# Autodesk Inventor assembly: Сборка ручка
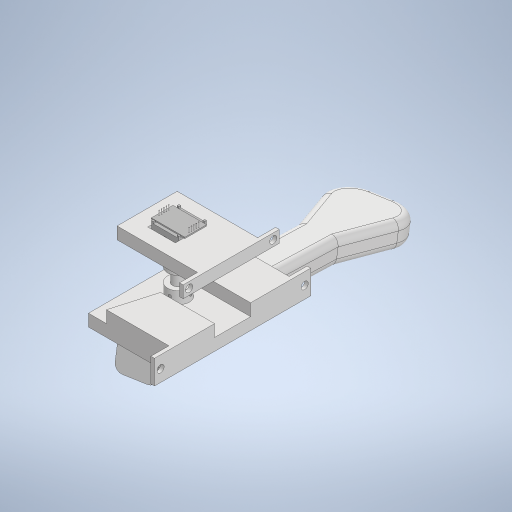
[picture p0: Inventor's stored thumbnail of the model, 512x512]
Saved by Autodesk Inventor 2023 (Build 270158000, 158)
## iProperties
Created: 2022-05-02
Part Number: Сборка ручка
Document SubType Name: Assembly
Designer: User
Author: User
## Documents named in this file (11)
- D:\Стойка\VR-simulator-3D-models\Механизм ручки\Сборка ручка.iam
- D:\Стойка\VR-simulator-3D-models\Механизм ручки\EAW.ipt
- D:\Стойка\VR-simulator-3D-models\Механизм ручки\Вал ручки.ipt
- D:\Стойка\VR-simulator-3D-models\Механизм ручки\Втулка энкодер.ipt
- D:\Стойка\VR-simulator-3D-models\Механизм ручки\Ручка.ipt
- D:\Стойка\VR-simulator-3D-models\Механизм ручки\Стенка.ipt
- D:\Стойка\VR-simulator-3D-models\Механизм ручки\Стопор.ipt
- D:\Стойка\VR-simulator-3D-models\Механизм ручки\Стенка энкодер.ipt
- D:\Стойка\VR-simulator-3D-models\Механизм ручки\Диск.ipt
- D:\Стойка\VR-simulator-3D-models\Механизм ручки\М3х8.ipt
- D:\Стойка\VR-simulator-3D-models\Механизм ручки\Шпилька.ipt
## Components (13 placed, 10 different names)
1. EAW:1 — Цилиндрический:4, Совмещение:15, Совмещение:18
2. Вал ручки:1 — Цилиндрический:13, Совмещение:13, Цилиндрический:14, Цилиндрический:15, Совмещение:19, Совмещение:21, Совмещение:22, Совмещение:23, Совмещение:25
3. Втулка энкодер:1 — Цилиндрический:4, Цилиндрический:15, Совмещение:19, Совмещение:20
4. Ручка:1 — Совмещение:23, Совмещение:24, Совмещение:26
5. Стенка:1 — Заподлицо:1, Цилиндрический:14, Совмещение:14
6. Стопор:1 — Цилиндрический:13, Совмещение:13, Совмещение:14
7. Стенка энкодер:1 — Заподлицо:1, Совмещение:15, Совмещение:18, Совмещение:20
8. М3х8:1 — Совмещение:21, Совмещение:25
9. Диск:2 — Цилиндрический:10, Совмещение:7, Совмещение:8
10. М3х8:2 — Цилиндрический:9, Цилиндрический:10, Совмещение:7, Совмещение:22
11. Диск:3 — Цилиндрический:8, Совмещение:9, Совмещение:10, Совмещение:26
12. М3х8:3 — Цилиндрический:7, Цилиндрический:8, Совмещение:10
13. Шпилька:1 — Цилиндрический:7, Цилиндрический:9, Совмещение:8, Совмещение:9, Совмещение:24
## Relationships (25: Mate 16, CylindricalJoint 8, Flush 1)
- Заподлицо:1 [Flush]: Стенка:1 ↔ Стенка энкодер:1
- Цилиндрический:4 [CylindricalJoint]: EAW:1 ↔ Втулка энкодер:1
- Цилиндрический:7 [CylindricalJoint]: М3х8:3 ↔ Шпилька:1
- Цилиндрический:8 [CylindricalJoint]: Диск:3 ↔ М3х8:3
- Цилиндрический:9 [CylindricalJoint]: М3х8:2 ↔ Шпилька:1
- Цилиндрический:10 [CylindricalJoint]: Диск:2 ↔ М3х8:2
- Совмещение:7 [Mate]: Диск:2 ↔ М3х8:2
- Совмещение:8 [Mate]: Диск:2 ↔ Шпилька:1
- Совмещение:9 [Mate]: Диск:3 ↔ Шпилька:1
- Совмещение:10 [Mate]: Диск:3 ↔ М3х8:3
- Цилиндрический:13 [CylindricalJoint]: Вал ручки:1 ↔ Стопор:1
- Совмещение:13 [Mate]: Вал ручки:1 ↔ Стопор:1
- Цилиндрический:14 [CylindricalJoint]: Вал ручки:1 ↔ Стенка:1
- Совмещение:14 [Mate]: Стенка:1 ↔ Стопор:1
- Совмещение:15 [Mate]: EAW:1 ↔ Стенка энкодер:1
- Совмещение:18 [Mate]: EAW:1 ↔ Стенка энкодер:1
- Цилиндрический:15 [CylindricalJoint]: Вал ручки:1 ↔ Втулка энкодер:1
- Совмещение:19 [Mate]: Вал ручки:1 ↔ Втулка энкодер:1
- Совмещение:20 [Mate]: Втулка энкодер:1 ↔ Стенка энкодер:1
- Совмещение:21 [Mate]: Вал ручки:1 ↔ М3х8:1
- Совмещение:22 [Mate]: Вал ручки:1 ↔ М3х8:2
- Совмещение:23 [Mate]: Вал ручки:1 ↔ Ручка:1
- Совмещение:24 [Mate]: Ручка:1 ↔ Шпилька:1
- Совмещение:25 [Mate]: Вал ручки:1 ↔ М3х8:1
- Совмещение:26 [Mate]: Ручка:1 ↔ Диск:3
